# Autodesk Inventor assembly: mobile_robot
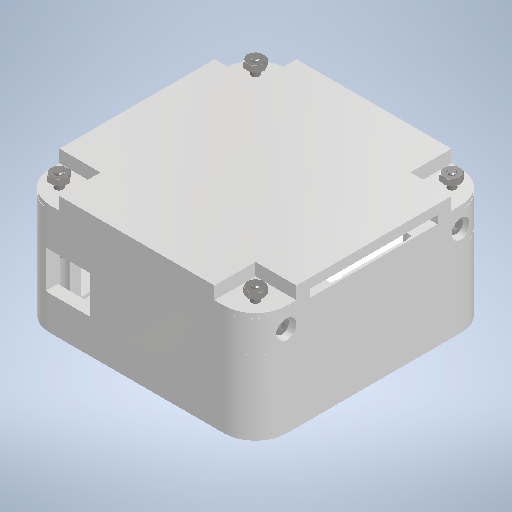
[picture p0: Inventor's stored thumbnail of the model, 512x512]
Saved by Autodesk Inventor 2025 (Build 290162000, 162)
## iProperties
Created: 2025-10-18
Part Number: mobile_robot
Document SubType Name: Assembly
Designer: sooo1
Author: sooo1
## Documents named in this file (18)
- C:\Users\sooo1\Documents\Inventor\MOBITOUCH\final\mobile_robot\mobile_robot.iam
- C:\Users\sooo1\Documents\Inventor\MOBITOUCH\final\mobile_robot\enclosure.ipt
- C:\Users\sooo1\Documents\Inventor\MOBITOUCH\final\mobile_robot\XL-320.ipt
- C:\Users\sooo1\Documents\Inventor\MOBITOUCH\final\mobile_robot\wheel.ipt
- C:\Users\sooo1\Documents\Inventor\MOBITOUCH\final\mobile_robot\tire_20-26.ipt
- C:\Users\sooo1\Documents\Inventor\MOBITOUCH\final\mobile_robot\odometry.ipt
- C:\Users\sooo1\Documents\Inventor\MOBITOUCH\final\mobile_robot\i2chub.ipt
- C:\Users\sooo1\Documents\Inventor\MOBITOUCH\final\mobile_robot\housing_motor.ipt
- C:\Users\sooo1\Documents\Inventor\MOBITOUCH\final\mobile_robot\lid.ipt
- C:\Users\sooo1\Documents\Inventor\MOBITOUCH\final\mobile_robot\opencm9.04.ipt
- C:\Users\sooo1\Documents\Inventor\MOBITOUCH\final\mobile_robot\plate_ball.ipt
- C:\Users\sooo1\Documents\Inventor\MOBITOUCH\final\mobile_robot\ball.ipt
- C:\Users\sooo1\Documents\Inventor\MOBITOUCH\final\mobile_robot\neodymiummagnet_Φ6.ipt
- C:\Users\sooo1\Documents\Inventor\MOBITOUCH\final\mobile_robot\JIS B 1176 - M2.5 x 20 - 0.45.ipt
- C:\Users\sooo1\Documents\Inventor\MOBITOUCH\final\mobile_robot\JIS B 1181 - M2.5.ipt
- C:\Users\sooo1\Documents\Inventor\MOBITOUCH\final\mobile_robot\JIS B 1176 - M2.5 x 16 - 0.45.ipt
- C:\Users\sooo1\Documents\Inventor\MOBITOUCH\final\mobile_robot\JIS B 1181 - M3.ipt
- C:\Users\sooo1\Documents\Inventor\MOBITOUCH\final\mobile_robot\JIS B 1176 - M3 x 16 - 0.5.ipt
## Components (36 placed, 17 different names)
1. enclosure:1 — フラッシュ:1, フラッシュ:2, フラッシュ:3, メイト:2, フラッシュ:4, メイト:4, メイト:13, メイト:15, メイト:17, メイト:18, メイト:19, メイト:20, メイト:22, メイト:48, メイト:50, メイト:55, メイト:56, メイト:57, メイト:58, メイト:59, メイト:60, メイト:61, メイト:62, メイト:63, メイト:64, メイト:65, メイト:66, 角度:2, メイト:75, メイト:77, メイト:78, メイト:80, メイト:81, メイト:82, メイト:83, メイト:97, メイト:99, メイト:100, メイト:101, メイト:102, メイト:103
2. XL-320:1 — メイト:1, メイト:2, メイト:3, メイト:7, メイト:8, メイト:9
3. XL-320:2 — フラッシュ:4, フラッシュ:5, メイト:4, メイト:10, メイト:11, メイト:12, 角度:3
4. wheel:1 — メイト:6, フラッシュ:7, メイト:7, メイト:8, メイト:9
5. wheel:2 — メイト:5, フラッシュ:6, メイト:10, メイト:11, メイト:12
6. tire_20-26:1 — メイト:6, フラッシュ:7, 正接:1
7. tire_20-26:2 — メイト:5, フラッシュ:6
8. odometry:1 — メイト:13, フラッシュ:8, メイト:16, メイト:75, 角度:3, メイト:106, メイト:107
9. i2chub:1 — メイト:15, フラッシュ:8, メイト:16
10. housing_motor:1 — メイト:17, メイト:18, メイト:19, メイト:21, メイト:76, メイト:79, メイト:92, メイト:93, メイト:94, メイト:95
11. lid:1 — メイト:20, メイト:21, メイト:22, メイト:88, メイト:89, メイト:90, メイト:91
12. opencm9.04:1 — メイト:48, メイト:49, メイト:50
13. plate_ball:1 — メイト:51, フラッシュ:9, メイト:52, メイト:57, メイト:58
14. ball:1 — メイト:51, フラッシュ:9, メイト:52
15. plate_ball:2 — メイト:55, メイト:56
16. ball:2
17. neodymiummagnet_Φ6:1 — メイト:59, メイト:63
18. neodymiummagnet_Φ6:2 — メイト:61, メイト:66
19. neodymiummagnet_Φ6:3 — メイト:62, メイト:65
20. neodymiummagnet_Φ6:4 — メイト:60, メイト:64
21. JIS B 1176 - メートル M2.5 x 20:1 — メイト:77, メイト:80, メイト:84
22. JIS B 1176 - メートル M2.5 x 20:2 — メイト:78, メイト:81, メイト:85
23. JIS B 1176 - メートル M2.5 x 20:3 — メイト:79, メイト:82, メイト:86
24. JIS B 1176 - メートル M2.5 x 20:4 — メイト:76, メイト:83, メイト:87
25. JIS B 1181 上 等級 2 - メートル 等級 2 上 M2.5:7 — メイト:84, メイト:90
26. JIS B 1181 上 等級 2 - メートル 等級 2 上 M2.5:8 — メイト:85, メイト:91
27. JIS B 1181 上 等級 2 - メートル 等級 2 上 M2.5:9 — メイト:87, メイト:89
28. JIS B 1181 上 等級 2 - メートル 等級 2 上 M2.5:10 — メイト:86, メイト:88
29. JIS B 1181 上 等級 2 - メートル 等級 2 上 M2.5:11 — メイト:96, メイト:97
30. JIS B 1181 上 等級 2 - メートル 等級 2 上 M2.5:12 — メイト:98, メイト:99
31. JIS B 1176 - メートル M2.5 x 16:1 — メイト:92, メイト:95, メイト:98
32. JIS B 1176 - メートル M2.5 x 16:2 — メイト:93, メイト:94, メイト:96
33. JIS B 1181 上 等級 2 - メートル 等級 2 上 M3:1 — メイト:105, メイト:107
34. JIS B 1181 上 等級 2 - メートル 等級 2 上 M3:2 — メイト:104, メイト:106
35. JIS B 1176 - メートル M3 x 16:1 — メイト:101, メイト:102, メイト:104
36. JIS B 1176 - メートル M3 x 16:2 — メイト:100, メイト:103, メイト:105
## Relationships (86: Mate 73, Flush 10, Angle 2, Tangent 1)
- フラッシュ:1 [Flush]: enclosure:1
- フラッシュ:2 [Flush]: enclosure:1
- フラッシュ:3 [Flush]: enclosure:1
- メイト:1 [Mate]: XL-320:1
- メイト:2 [Mate]: enclosure:1 ↔ XL-320:1
- フラッシュ:4 [Flush]: enclosure:1 ↔ XL-320:2
- メイト:3 [Mate]: XL-320:1
- フラッシュ:5 [Flush]: XL-320:2
- メイト:4 [Mate]: enclosure:1 ↔ XL-320:2
- メイト:5 [Mate]: wheel:2 ↔ tire_20-26:2
- メイト:6 [Mate]: wheel:1 ↔ tire_20-26:1
- フラッシュ:6 [Flush]: wheel:2 ↔ tire_20-26:2
- フラッシュ:7 [Flush]: wheel:1 ↔ tire_20-26:1
- メイト:7 [Mate]: XL-320:1 ↔ wheel:1
- メイト:8 [Mate]: XL-320:1 ↔ wheel:1
- メイト:9 [Mate]: XL-320:1 ↔ wheel:1
- メイト:10 [Mate]: XL-320:2 ↔ wheel:2
- メイト:11 [Mate]: XL-320:2 ↔ wheel:2
- メイト:12 [Mate]: XL-320:2 ↔ wheel:2
- メイト:13 [Mate]: enclosure:1 ↔ odometry:1
- メイト:15 [Mate]: enclosure:1 ↔ i2chub:1
- フラッシュ:8 [Flush]: odometry:1 ↔ i2chub:1
- メイト:16 [Mate]: odometry:1 ↔ i2chub:1
- メイト:17 [Mate]: enclosure:1 ↔ housing_motor:1
- メイト:18 [Mate]: enclosure:1 ↔ housing_motor:1
- メイト:19 [Mate]: enclosure:1 ↔ housing_motor:1
- メイト:20 [Mate]: enclosure:1 ↔ lid:1
- メイト:21 [Mate]: housing_motor:1 ↔ lid:1
- メイト:22 [Mate]: enclosure:1 ↔ lid:1
- メイト:48 [Mate]: enclosure:1 ↔ opencm9.04:1
- メイト:49 [Mate]: opencm9.04:1
- メイト:50 [Mate]: enclosure:1 ↔ opencm9.04:1
- メイト:51 [Mate]: plate_ball:1 ↔ ball:1
- フラッシュ:9 [Flush]: plate_ball:1 ↔ ball:1
- メイト:52 [Mate]: plate_ball:1 ↔ ball:1
- [Mate]: plate_ball:2 ↔ ball:2
- [Flush]: plate_ball:2 ↔ ball:2
- [Mate]: plate_ball:2 ↔ ball:2
- メイト:55 [Mate]: enclosure:1 ↔ plate_ball:2
- メイト:56 [Mate]: enclosure:1 ↔ plate_ball:2
- メイト:57 [Mate]: enclosure:1 ↔ plate_ball:1
- メイト:58 [Mate]: enclosure:1 ↔ plate_ball:1
- メイト:59 [Mate]: enclosure:1 ↔ neodymiummagnet_Φ6:1
- メイト:60 [Mate]: enclosure:1 ↔ neodymiummagnet_Φ6:4
- メイト:61 [Mate]: enclosure:1 ↔ neodymiummagnet_Φ6:2
- メイト:62 [Mate]: enclosure:1 ↔ neodymiummagnet_Φ6:3
- メイト:63 [Mate]: enclosure:1 ↔ neodymiummagnet_Φ6:1
- メイト:64 [Mate]: enclosure:1 ↔ neodymiummagnet_Φ6:4
- メイト:65 [Mate]: enclosure:1 ↔ neodymiummagnet_Φ6:3
- メイト:66 [Mate]: enclosure:1 ↔ neodymiummagnet_Φ6:2
- 角度:2 [Angle] (0 deg): enclosure:1
- 正接:1 [Tangent]: tire_20-26:1
- メイト:75 [Mate]: enclosure:1 ↔ odometry:1
- 角度:3 [Angle] (180 deg): XL-320:2 ↔ odometry:1
- メイト:76 [Mate]: housing_motor:1 ↔ JIS B 1176 - メートル M2.5 x 20:4
- メイト:77 [Mate]: enclosure:1 ↔ JIS B 1176 - メートル M2.5 x 20:1
- メイト:78 [Mate]: enclosure:1 ↔ JIS B 1176 - メートル M2.5 x 20:2
- メイト:79 [Mate]: housing_motor:1 ↔ JIS B 1176 - メートル M2.5 x 20:3
- メイト:80 [Mate]: enclosure:1 ↔ JIS B 1176 - メートル M2.5 x 20:1
- メイト:81 [Mate]: enclosure:1 ↔ JIS B 1176 - メートル M2.5 x 20:2
- メイト:82 [Mate]: enclosure:1 ↔ JIS B 1176 - メートル M2.5 x 20:3
- メイト:83 [Mate]: enclosure:1 ↔ JIS B 1176 - メートル M2.5 x 20:4
- メイト:84 [Mate]: JIS B 1176 - メートル M2.5 x 20:1 ↔ JIS B 1181 上 等級 2 - メートル 等級 2 上 M2.5:7
- メイト:85 [Mate]: JIS B 1176 - メートル M2.5 x 20:2 ↔ JIS B 1181 上 等級 2 - メートル 等級 2 上 M2.5:8
- メイト:86 [Mate]: JIS B 1176 - メートル M2.5 x 20:3 ↔ JIS B 1181 上 等級 2 - メートル 等級 2 上 M2.5:10
- メイト:87 [Mate]: JIS B 1176 - メートル M2.5 x 20:4 ↔ JIS B 1181 上 等級 2 - メートル 等級 2 上 M2.5:9
- メイト:88 [Mate] (2 mm): lid:1 ↔ JIS B 1181 上 等級 2 - メートル 等級 2 上 M2.5:10
- メイト:89 [Mate] (2 mm): lid:1 ↔ JIS B 1181 上 等級 2 - メートル 等級 2 上 M2.5:9
- メイト:90 [Mate] (2 mm): lid:1 ↔ JIS B 1181 上 等級 2 - メートル 等級 2 上 M2.5:7
- メイト:91 [Mate] (2 mm): lid:1 ↔ JIS B 1181 上 等級 2 - メートル 等級 2 上 M2.5:8
- メイト:92 [Mate]: housing_motor:1 ↔ JIS B 1176 - メートル M2.5 x 16:1
- メイト:93 [Mate]: housing_motor:1 ↔ JIS B 1176 - メートル M2.5 x 16:2
- メイト:94 [Mate]: housing_motor:1 ↔ JIS B 1176 - メートル M2.5 x 16:2
- メイト:95 [Mate]: housing_motor:1 ↔ JIS B 1176 - メートル M2.5 x 16:1
- メイト:96 [Mate]: JIS B 1181 上 等級 2 - メートル 等級 2 上 M2.5:11 ↔ JIS B 1176 - メートル M2.5 x 16:2
- メイト:97 [Mate]: enclosure:1 ↔ JIS B 1181 上 等級 2 - メートル 等級 2 上 M2.5:11
- メイト:98 [Mate]: JIS B 1181 上 等級 2 - メートル 等級 2 上 M2.5:12 ↔ JIS B 1176 - メートル M2.5 x 16:1
- メイト:99 [Mate]: enclosure:1 ↔ JIS B 1181 上 等級 2 - メートル 等級 2 上 M2.5:12
- メイト:100 [Mate]: enclosure:1 ↔ JIS B 1176 - メートル M3 x 16:2
- メイト:101 [Mate]: enclosure:1 ↔ JIS B 1176 - メートル M3 x 16:1
- メイト:102 [Mate]: enclosure:1 ↔ JIS B 1176 - メートル M3 x 16:1
- メイト:103 [Mate]: enclosure:1 ↔ JIS B 1176 - メートル M3 x 16:2
- メイト:104 [Mate]: JIS B 1181 上 等級 2 - メートル 等級 2 上 M3:2 ↔ JIS B 1176 - メートル M3 x 16:1
- メイト:105 [Mate]: JIS B 1181 上 等級 2 - メートル 等級 2 上 M3:1 ↔ JIS B 1176 - メートル M3 x 16:2
- メイト:106 [Mate]: odometry:1 ↔ JIS B 1181 上 等級 2 - メートル 等級 2 上 M3:2
- メイト:107 [Mate]: odometry:1 ↔ JIS B 1181 上 等級 2 - メートル 等級 2 上 M3:1
## Named parameters: d87_d84 = 0 mm, d88_d85 = 0 mm, d89_d86 = 0 mm
